# Autodesk Inventor assembly: A2017_T5_02
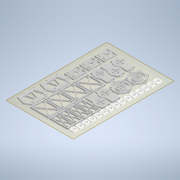
[picture p0: Inventor's stored thumbnail of the model, 180x180]
Saved by Autodesk Inventor 2020 (Build 240168000, 168)
## iProperties
Created: 2021-08-27
Part Number: A2017_T5_02
Document SubType Name: Assembly
Designer: Masato
Author: Masato
## Documents named in this file (10)
- C:\Users\L20C1118 森　圭汰\Documents\2022_0321_open\SUSTAINA-OP\Cam\A2017_T5_02.iam
- C:\Users\L20C1118 森　圭汰\Documents\2022_0321_open\SUSTAINA-OP\Cam\DisposableBoard.ipt
- C:\Users\L20C1118 森　圭汰\Documents\2022_0321_open\SUSTAINA-OP\LowerBody\Knee\Knee_clamp.ipt
- C:\Users\L20C1118 森　圭汰\Documents\2022_0321_open\SUSTAINA-OP\UpperBody\Trunk\Trunk_lower_side_frame.ipt
- C:\Users\L20C1118 森　圭汰\Documents\2022_0321_open\SUSTAINA-OP\UpperBody\Arm\Shoulder_horn_frame.ipt
- C:\Users\L20C1118 森　圭汰\Documents\2022_0321_open\SUSTAINA-OP\LowerBody\Link\FrontLink_diagonal.ipt
- C:\Users\L20C1118 森　圭汰\Documents\2022_0321_open\SUSTAINA-OP\LowerBody\Link\BackLink_diagonal.ipt
- C:\Users\L20C1118 森　圭汰\Documents\2022_0321_open\SUSTAINA-OP\LowerBody\Leg_joint\Leg_joint_yaw_frame.ipt
- C:\Users\L20C1118 森　圭汰\Documents\2022_0321_open\SUSTAINA-OP\UpperBody\Trunk\CrossRollerBearing\Inner_support_stand.ipt
- C:\Users\L20C1118 森　圭汰\Documents\2022_0321_open\SUSTAINA-OP\UpperBody\Trunk\CrossRollerBearing\Outer_support_stand.ipt
## Components (38 placed, 9 different names)
1. DisposableBoard:1 — メイト:2, メイト:1, フラッシュ:1, フラッシュ:2, メイト:4, メイト:5, メイト:6, メイト:7, メイト:8, フラッシュ:4, フラッシュ:7, 正接:1, 角度:1, フラッシュ:8, 正接:2, メイト:14, メイト:15, メイト:18, メイト:19, メイト:20, メイト:21, 角度:2, 角度:3, 角度:4, 角度:5, メイト:23, メイト:24, メイト:25
2. Leg_joint_yaw_frame:1 — メイト:15, フラッシュ:9, 正接:5, 正接:7, 正接:9, 正接:10
3. Leg_joint_yaw_frame:2 — メイト:14, メイト:16, フラッシュ:9, 正接:4, 正接:5
4. Inner_support_stand:1 — メイト:21, 正接:11, 角度:4
5. Inner_support_stand:2 — メイト:18, 正接:12, 角度:5
6. Outer_support_stand:1 — メイト:20, 角度:3, 正接:8, 正接:10, 正接:12
7. Outer_support_stand:2 — メイト:19, 角度:2, 正接:7, 正接:8, 正接:9, 正接:11
8. Leg_joint_yaw_frame:3 — メイト:23, 正接:14, フラッシュ:12, フラッシュ:13, 正接:15
9. Leg_joint_yaw_frame:4 — メイト:24, フラッシュ:13, 正接:15, フラッシュ:14, 正接:16
10. Leg_joint_yaw_frame:5 — メイト:25, フラッシュ:14, 正接:16
11. FrontLink_diagonal:1 — メイト:6, フラッシュ:4, メイト:10, メイト:12
12. FrontLink_diagonal:2
13. FrontLink_diagonal:3 — メイト:16
14. FrontLink_diagonal:4 — メイト:22, 正接:14, フラッシュ:12
15. BackLink_diagonal:1 — メイト:5, メイト:10, フラッシュ:7, 正接:3
16. BackLink_diagonal:2
17. BackLink_diagonal:3
18. BackLink_diagonal:4 — 正接:4
19. Trunk_lower_side_frame:1 — メイト:4, メイト:12, 正接:1, フラッシュ:8
20. Trunk_lower_side_frame:2 — 正接:6, 正接:13
21. Knee_clamp:1 — メイト:7, 角度:1, 正接:2, 正接:3
22. Knee_clamp:2
23. Knee_clamp:3
24. Knee_clamp:4
25. Knee_clamp:5
26. Knee_clamp:6
27. Knee_clamp:7
28. Knee_clamp:8
29. Knee_clamp:9
30. Knee_clamp:10
31. Knee_clamp:11
32. Knee_clamp:12
33. Knee_clamp:13
34. Knee_clamp:14
35. Knee_clamp:15
36. Shoulder_horn_frame:1 — メイト:8, 正接:6, 正接:13, メイト:22
37. Shoulder_horn_frame:2
38. Shoulder_horn_frame:3
## Component patterns: (4 elements, first: FrontLink_diagonal:1), (4 elements, first: BackLink_diagonal:1), (2 elements, first: Trunk_lower_side_frame:1), (15 elements, first: Knee_clamp:1), (3 elements, first: Shoulder_horn_frame:1)
## Relationships (50: Mate 20, Tangent 16, Flush 9, Angle 5)
- メイト:2 [Mate]: DisposableBoard:1
- メイト:1 [Mate]: DisposableBoard:1
- フラッシュ:1 [Flush]: DisposableBoard:1
- フラッシュ:2 [Flush]: DisposableBoard:1
- メイト:4 [Mate]: DisposableBoard:1 ↔ Trunk_lower_side_frame:1
- メイト:5 [Mate]: DisposableBoard:1 ↔ BackLink_diagonal:1
- メイト:6 [Mate]: DisposableBoard:1 ↔ FrontLink_diagonal:1
- メイト:7 [Mate]: DisposableBoard:1 ↔ Knee_clamp:1
- メイト:8 [Mate]: DisposableBoard:1 ↔ Shoulder_horn_frame:1
- フラッシュ:4 [Flush] (2 mm): DisposableBoard:1 ↔ FrontLink_diagonal:1
- メイト:10 [Mate] (2.5 mm): FrontLink_diagonal:1 ↔ BackLink_diagonal:1
- フラッシュ:7 [Flush] (2 mm): DisposableBoard:1 ↔ BackLink_diagonal:1
- メイト:12 [Mate] (2.5 mm): FrontLink_diagonal:1 ↔ Trunk_lower_side_frame:1
- 正接:1 [Tangent] (2 mm): DisposableBoard:1 ↔ Trunk_lower_side_frame:1
- 角度:1 [Angle] (45 deg): DisposableBoard:1 ↔ Knee_clamp:1
- フラッシュ:8 [Flush] (2 mm): DisposableBoard:1 ↔ Trunk_lower_side_frame:1
- 正接:2 [Tangent] (2 mm): DisposableBoard:1 ↔ Knee_clamp:1
- 正接:3 [Tangent] (3.4 mm): BackLink_diagonal:1 ↔ Knee_clamp:1
- メイト:14 [Mate]: DisposableBoard:1 ↔ Leg_joint_yaw_frame:2
- メイト:15 [Mate]: DisposableBoard:1 ↔ Leg_joint_yaw_frame:1
- メイト:16 [Mate] (2.5 mm): Leg_joint_yaw_frame:2 ↔ FrontLink_diagonal:3
- フラッシュ:9 [Flush]: Leg_joint_yaw_frame:1 ↔ Leg_joint_yaw_frame:2
- 正接:4 [Tangent] (2.5 mm): Leg_joint_yaw_frame:2 ↔ BackLink_diagonal:4
- 正接:5 [Tangent] (3 mm): Leg_joint_yaw_frame:1 ↔ Leg_joint_yaw_frame:2
- メイト:18 [Mate]: DisposableBoard:1 ↔ Inner_support_stand:2
- メイト:19 [Mate]: DisposableBoard:1 ↔ Outer_support_stand:2
- メイト:20 [Mate]: DisposableBoard:1 ↔ Outer_support_stand:1
- メイト:21 [Mate]: DisposableBoard:1 ↔ Inner_support_stand:1
- 正接:6 [Tangent] (2.5 mm): Trunk_lower_side_frame:2 ↔ Shoulder_horn_frame:1
- 角度:2 [Angle] (30 deg): DisposableBoard:1 ↔ Outer_support_stand:2
- 角度:3 [Angle] (30 deg): DisposableBoard:1 ↔ Outer_support_stand:1
- 正接:7 [Tangent] (2.5 mm): Leg_joint_yaw_frame:1 ↔ Outer_support_stand:2
- 正接:8 [Tangent] (2.5 mm): Outer_support_stand:1 ↔ Outer_support_stand:2
- 正接:9 [Tangent]: Leg_joint_yaw_frame:1 ↔ Outer_support_stand:2
- 正接:10 [Tangent]: Leg_joint_yaw_frame:1 ↔ Outer_support_stand:1
- 正接:11 [Tangent] (-4 mm): Inner_support_stand:1 ↔ Outer_support_stand:2
- 正接:12 [Tangent] (-4 mm): Inner_support_stand:2 ↔ Outer_support_stand:1
- 角度:4 [Angle] (0 deg): DisposableBoard:1 ↔ Inner_support_stand:1
- 角度:5 [Angle] (0 deg): DisposableBoard:1 ↔ Inner_support_stand:2
- 正接:13 [Tangent] (2.5 mm): Trunk_lower_side_frame:2 ↔ Shoulder_horn_frame:1
- メイト:22 [Mate] (6.9 mm): FrontLink_diagonal:4 ↔ Shoulder_horn_frame:1
- メイト:23 [Mate]: DisposableBoard:1 ↔ Leg_joint_yaw_frame:3
- 正接:14 [Tangent] (2.5 mm): Leg_joint_yaw_frame:3 ↔ FrontLink_diagonal:4
- フラッシュ:12 [Flush]: Leg_joint_yaw_frame:3 ↔ FrontLink_diagonal:4
- メイト:24 [Mate]: DisposableBoard:1 ↔ Leg_joint_yaw_frame:4
- フラッシュ:13 [Flush]: Leg_joint_yaw_frame:3 ↔ Leg_joint_yaw_frame:4
- 正接:15 [Tangent] (2.5 mm): Leg_joint_yaw_frame:3 ↔ Leg_joint_yaw_frame:4
- メイト:25 [Mate]: DisposableBoard:1 ↔ Leg_joint_yaw_frame:5
- フラッシュ:14 [Flush]: Leg_joint_yaw_frame:4 ↔ Leg_joint_yaw_frame:5
- 正接:16 [Tangent] (2.5 mm): Leg_joint_yaw_frame:4 ↔ Leg_joint_yaw_frame:5
